# Autodesk Inventor assembly: wheelAssembly
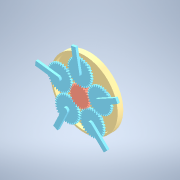
[picture p0: Inventor's stored thumbnail of the model, 180x180]
Saved by Autodesk Inventor 2020.1 (Build 241239000, 239)
## iProperties
Created: 2020-01-18
Part Number: wheelAssembly
Document SubType Name: Assembly
Designer: Ali
Author: Ali
## Documents named in this file (7)
- F:\Inventor_Projects\AlorsBot_CAD\inventor\assemblies\wheelAssembly.iam
- F:\Inventor_Projects\AlorsBot_CAD\inventor\parts\wheel.ipt
- F:\Inventor_Projects\AlorsBot_CAD\inventor\parts\innerGear.ipt
- F:\Inventor_Projects\AlorsBot_CAD\inventor\parts\outerGear.ipt
- F:\Inventor_Projects\AlorsBot_CAD\inventor\parts\bearing.ipt
- F:\Inventor_Projects\AlorsBot_CAD\inventor\parts\block.ipt
- F:\Inventor_Projects\AlorsBot_CAD\inventor\excel\wheelParameters.xlsx
## Components (9 placed, 5 different names)
1. wheel:1 — Insert:3, Mate:2, Mate:3, Mate:4, Insert:4, Mate:7, Insert:5
2. innerGear:1 — Insert:5
3. bearing:1 — Insert:3
4. block:1 — Mate:5, Mate:6
5. outerGear:1 — Insert:4
6. outerGear:2
7. outerGear:3
8. outerGear:4
9. outerGear:5
## Component patterns: (5 elements, first: outerGear:1)
## Relationships (9: Mate 6, Insert 3)
- Insert:3: wheel:1 ↔ bearing:1
- Mate:2: wheel:1
- Mate:3: wheel:1
- Mate:4: wheel:1
- Mate:5 (-1.9 mm): block:1
- Mate:6 (7.1 mm): block:1
- Insert:4 (-3 mm): wheel:1 ↔ outerGear:1
- Mate:7: wheel:1
- Insert:5: wheel:1 ↔ innerGear:1
## Named parameters: Wheel_Related_W_ = 0, W_innerDiameter = 70 mm, W_innerDepth = 4 mm, W_wallThickness = 2 mm, W_holesClearance = 0.3 mm, W_outerGearHoleDiameter = 5.3 mm, W_innerGearHoleDiameter = 10.1 mm, TempSpotReserved7 = 0 mm, TempSpotReserved8 = 0 mm, TempSpotReserved9 = 0 mm, TempSpotReserved10 = 0 mm, TempSpotReserved11 = 0 mm, TempSpotReserved12 = 0 mm, TempSpotReserved13 = 0 mm, TempSpotReserved14 = 0 mm, TempSpotReserved15 = 0 mm, TempSpotReserved16 = 0 mm, TempSpotReserved17 = 0 mm, TempSpotReserved18 = 0 mm, TempSpotReserved19 = 0 mm, TempSpotReserved20 = 0 mm, Inner_Gear_Related_IG_ = 0, IG_shaftDiameter = 7.5 mm, IG_gearDiameter = 20 mm, IG_shaftLength = 17 mm, IG_gearThickness = 2 mm, TempSpotReserved25 = 0 mm, TempSpotReserved26 = 0 mm, TempSpotReserved27 = 0 mm, TempSpotReserved28 = 0 mm, TempSpotReserved29 = 0 mm, TempSpotReserved30 = 0 mm, TempSpotReserved31 = 0 mm, TempSpotReserved32 = 0 mm, TempSpotReserved33 = 0 mm, TempSpotReserved34 = 0 mm, TempSpotReserved35 = 0 mm, TempSpotReserved36 = 0 mm, TempSpotReserved37 = 0 mm, TempSpotReserved38 = 0 mm, TempSpotReserved39 = 0 mm, TempSpotReserved40 = 0 mm, Outer_Gear_Related_OG_ = 0, OG_distanceFromCenter = 22.5 mm, OG_shaftDiameter = 5 mm, OG_gearDiameter = 25 mm, OG_numberOfGears = 5, OG_shaftLength = 9 mm, OG_gearThickness = 2 mm, TempSpotReserved47 = 0 mm, TempSpotReserved48 = 0 mm, TempSpotReserved49 = 0 mm, TempSpotReserved50 = 0 mm, TempSpotReserved51 = 0 mm, TempSpotReserved52 = 0 mm, TempSpotReserved53 = 0 mm, TempSpotReserved54 = 0 mm, TempSpotReserved55 = 0 mm, TempSpotReserved56 = 0 mm, TempSpotReserved57 = 0 mm, TempSpotReserved58 = 0 mm, TempSpotReserved59 = 0 mm, TempSpotReserved60 = 0 mm, Leg_Extensions_Related_LE_ = 0, LE_baseDiameter = 5 mm, LE_maxLength = 23.67256 mm, LE_thickness = 2.5 mm, IG_ratioToOuterGear = 1.25, B_bearingThickness = 1 mm, TempSpotReserved43 = 0 mm, TempSpotReserved45 = 0 mm, Thisisatest = 25.4 mm, TempSpotReserved46 = 0 mm, TempSpotReserved44 = 0 mm, LE_offsetAboveOuterGear = 0 mm, Bearing_Related_B_ = 0, TempSpotReserved42 = 0 mm, OG_skirtOffset = 5 mm, OG_skirtThickness = 1 mm, IG_skirtThickness = 2 mm, IG_skirtOffset = 10 mm, IG_extentionLength = 19.5 mm, IG_extentionThickness = 3 mm, IG_slitWidth = 4 mm, IG_slitlength = 8 mm, IG_slitDistanceFromCenterHole = 7 mm, IG_slitClearance = 0.2 mm, Reserved_10 = 0 mm, Reserved_9 = 0 mm, Reserved_11 = 0 mm, Reserved_12 = 0 mm, Reserved_8 = 0 mm, Reserved_7 = 0 mm, Reserved_26 = 0 mm, Reserved_20 = 0 mm, Reserved_22 = 0 mm, Reserved_23 = 0 mm, Reserved_25 = 0 mm, Reserved_24 = 0 mm, Reserved_21 = 0 mm, Reserved_19 = 0 mm, Reserved_27 = 0 mm, Reserved_14 = 0 mm, Reserved_15 = 0 mm, Reserved_16 = 0 mm, Reserved_13 = 0 mm, Reserved_17 = 0 mm, Reserved_18 = 0 mm, Bearing_Related_BR_ = 0, BR_bearingThickness = 1 mm, Block_Related_BL_ = 0, BL_width = 3.8 mm, BL_length = 7.8 mm, BL_depth = 10 mm, W_filletRadius = 0.25 mm, W_numberOfSlits = 4, W_extrutsionTaperAngle = 2 deg, OG_protrudeDistance = 3 mm, IG_dAxleDepth = 5 mm, IG_dAxleShort = 1.5 mm, IG_dAxleCircleDiameter = 2 mm, IG_gearRatio = 1.25
